# Autodesk Inventor assembly: Cover-Plate-short-with-bolts
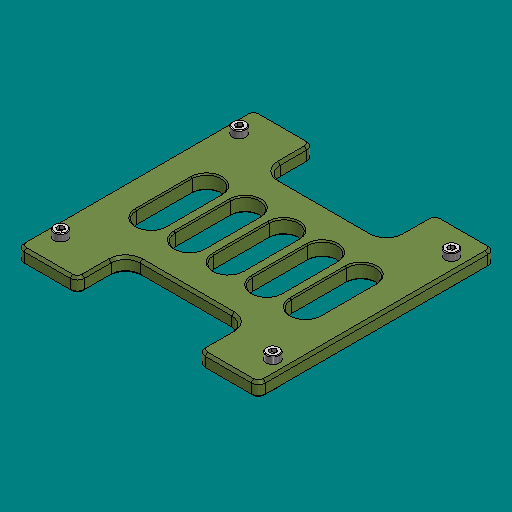
[picture p0: Inventor's stored thumbnail of the model, 512x512]
Saved by Autodesk Inventor 2025 (Build 290162000, 162)
## iProperties
Created: 2024-07-04
Part Number: Cover-Plate-short-with-bolts
Document SubType Name: Assembly
Designer: kuzmin
Author: kuzmin
## Documents named in this file (3)
- C:\Users\queez\Dropbox\Drawings\PIHTI\Plasma Vessel\Cathode-Flange-Cage\Cover-Plate-short-with-bolts.iam
- C:\Users\queez\Dropbox\Drawings\PIHTI\Plasma Vessel\Cathode-Flange-Cage\Cover-Plate-short-with-holes.ipt
- C:\Users\queez\Dropbox\Drawings\PIHTI\ContentCenter\Fastners\M3x10-SHCS.ipt
## Components (5 placed, 2 different names)
1. Cover-Plate-short-with-holes:1
2. JIS B 1176 - Metric M3 x 10:1
3. JIS B 1176 - Metric M3 x 10:2
4. JIS B 1176 - Metric M3 x 10:3
5. JIS B 1176 - Metric M3 x 10:4
## Relationships (4: WeldJoint 4)
- [WeldJoint]: Cover-Plate-short-with-holes:1 ↔ JIS B 1176 - Metric M3 x 10:1
- [WeldJoint]: Cover-Plate-short-with-holes:1 ↔ JIS B 1176 - Metric M3 x 10:3
- [WeldJoint]: Cover-Plate-short-with-holes:1 ↔ JIS B 1176 - Metric M3 x 10:2
- [WeldJoint]: Cover-Plate-short-with-holes:1 ↔ JIS B 1176 - Metric M3 x 10:4
